# Autodesk Inventor assembly: Assembly
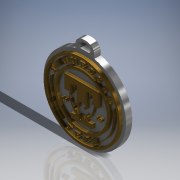
[picture p0: Inventor's stored thumbnail of the model, 180x180]
Saved by Autodesk Inventor 2018 (Build 220112000, 112)
## iProperties
Created: 2017-11-28
Part Number: Assembly
Document SubType Name: Assembly
Designer: Rus
Author: Rus
## Documents named in this file (3)
- E:\Libraries\Documents\3D Models\2017 TN Tech Ornament\Assembly.iam
- E:\Libraries\Documents\3D Models\2017 TN Tech Ornament\Aluminum Backing.ipt
- E:\Libraries\Documents\3D Models\2017 TN Tech Ornament\Brass Logo.ipt
## Components (2 placed, 2 different names)
1. Aluminum Backing:1 — Angle:1, Flush:2, Mate:2
2. Brass Logo:1 — Flush:1, Angle:1, Mate:1
## Relationships (6: Mate 3, Flush 2, Angle 1)
- Flush:1 (-3.175 mm): Brass Logo:1
- Angle:1 (0 deg): Aluminum Backing:1 ↔ Brass Logo:1
- Flush:2: Aluminum Backing:1
- Mate:1: Brass Logo:1
- Mate:2: Aluminum Backing:1
- Mate:3
